# Autodesk Inventor assembly: California_Corner_MIR
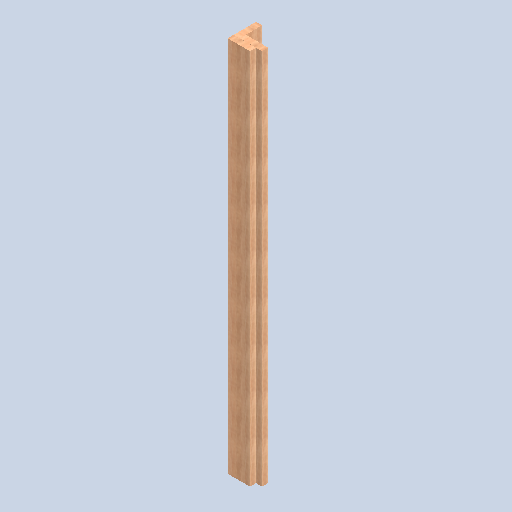
[picture p0: Inventor's stored thumbnail of the model, 512x512]
Saved by Autodesk Inventor 2025 (Build 290162010, 162A)
## iProperties
Created: 2024-09-15
Part Number: California_Corner_MIR
Document SubType Name: Assembly
Designer: Tom
Author: Tom
## Documents named in this file (2)
- C:\Users\Tom\Documents\Inventor\Mobility\Additional_Building\California_Corner_MIR.iam
- C:\Users\Tom\Documents\Inventor\Mobility\Additional_Building\Stud_MIR.ipt
## Components (3 placed, 1 different names)
1. Stud_MIR:1 — Flush:2, Flush:1, Mate:1, Flush:3, Mate:3
2. Stud_MIR:2 — Flush:2, Flush:1, Mate:1, Mate:2
3. Stud_MIR:3 — Flush:3, Mate:3, Mate:2
## Relationships (6: Flush 3, Mate 3)
- Flush:2: Stud_MIR:1 ↔ Stud_MIR:2
- Flush:1: Stud_MIR:1 ↔ Stud_MIR:2
- Mate:1: Stud_MIR:1 ↔ Stud_MIR:2
- Flush:3: Stud_MIR:1 ↔ Stud_MIR:3
- Mate:3: Stud_MIR:1 ↔ Stud_MIR:3
- Mate:2: Stud_MIR:2 ↔ Stud_MIR:3
